# Autodesk Inventor assembly: mock up 1
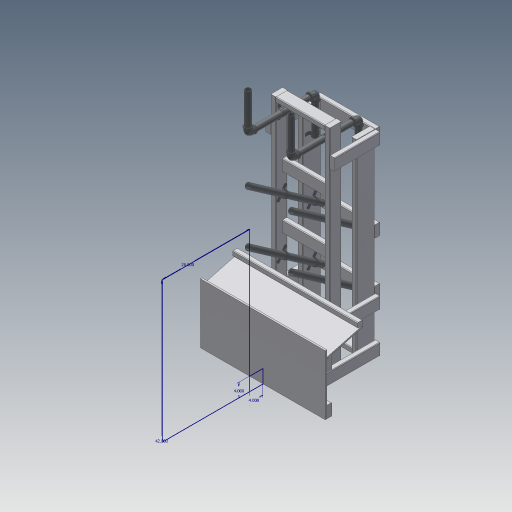
[picture p0: Inventor's stored thumbnail of the model, 512x512]
Saved by Autodesk Inventor 2023.5 (Build 275446000, 446)
## iProperties
Created: 2025-01-04
Part Number: mock up 1
Document SubType Name: Assembly
Designer: BAM
Author: BAM
## Documents named in this file (3)
- C:\Users\BAM\Documents\GitHub\2025-ReefScape---CAD\mock up 1.iam
- C:\Users\BAM\Documents\GitHub\2025-ReefScape---CAD\Field Items\TE-25300\TE-25300.iam
- C:\Users\BAM\Documents\GitHub\2025-ReefScape---CAD\mock up sketch 1.ipt
## Components (2 placed, 2 different names)
1. TE-25300:1 [sub-assembly] — Mate:1, Mate:2
2. mock up sketch 1:1 — Flush:2, Mate:1, Mate:2
## Relationships (3: Mate 2, Flush 1)
- Flush:2: mock up sketch 1:1
- Mate:1: TE-25300:1 ↔ mock up sketch 1:1
- Mate:2: TE-25300:1 ↔ mock up sketch 1:1
